# Autodesk Inventor assembly: Base
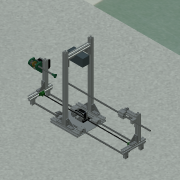
[picture p0: Inventor's stored thumbnail of the model, 180x180]
Saved by Autodesk Inventor 2015 (Build 190159000, 159)
## iProperties
Created: 2015-02-24
Part Number: Base
Document SubType Name: Assembly
Designer: Andrew
Author: Andrew
## Documents named in this file (33)
- C:\Users\pltwe4\Documents\model\Base.iam
- C:\Users\pltwe4\Documents\model\Linear Bearing Platform Small.ipt
- C:\Users\pltwe4\Documents\model\Base Plate.ipt
- C:\Users\pltwe4\Documents\model\NEMA 17 Stepper.ipt
- C:\Users\pltwe4\Documents\model\GT2 Pulley.ipt
- C:\Users\pltwe4\Documents\model\Stepper Motor Mount.ipt
- C:\Users\pltwe4\Documents\model\MainRod.ipt
- C:\Users\pltwe4\Documents\model\Linear Rail Shaft Guide.ipt
- C:\Users\pltwe4\Documents\model\Spur Gear.ipt
- C:\Users\pltwe4\Documents\model\Worm Gear.ipt
- C:\Users\pltwe4\Documents\model\20x20 Slotted Extrusion Arm.ipt
- C:\Users\pltwe4\Documents\model\20x20 Slotted Extrusion Tower.ipt
- C:\Users\pltwe4\Documents\model\Corner Brace.ipt
- C:\Users\pltwe4\Documents\model\Stepper Gear Box.ipt
- C:\Users\pltwe4\Documents\model\Bearing.ipt
- C:\Users\pltwe4\Documents\model\20x20 Slotted Extrusion Stationary Arm.ipt
- C:\Users\pltwe4\Documents\model\Clamp Rod.ipt
- C:\Users\pltwe4\Documents\model\Rotational Rod.ipt
- C:\Users\pltwe4\Documents\model\20x20 Slotted Extrusion Base.ipt
- C:\Users\pltwe4\Documents\model\20x20 Slotted Extrusion Source Bracket.ipt
- C:\Users\pltwe4\Documents\model\Cover.ipt
- C:\Users\pltwe4\Documents\model\X-Ray Tube Assy.ipt.iam
- C:\Users\pltwe4\Documents\model\Hand.ipt
- C:\Users\pltwe4\Documents\model\Linear Bearing Adapter Arm.ipt
- C:\Users\pltwe4\Documents\model\20x20 Slotted Extrusion Base2Plate.ipt
- C:\Users\pltwe4\Documents\model\UnNeeded\Corner Brace_MIR.ipt
- C:\Users\pltwe4\Documents\model\Stepper Adapter.ipt
- C:\Users\pltwe4\Documents\model\Stepper Adapter Cap.ipt
- C:\Users\pltwe4\Documents\model\Belt Clamp.ipt
- C:\Users\pltwe4\Documents\model\GT2 Belt Cut.ipt
- C:\Users\pltwe4\Documents\model\Limit Adapter.ipt
- C:\Users\pltwe4\Documents\model\Limit Switch.ipt
- X-Ray Tube Assy.ipt
## Components (194 placed, 31 different names)
1. Linear Bearing Platform Small:1 — Flush:5, Mate:7, Flush:9, Flush:11
2. Linear Bearing Platform Small:2 — Flush:4, Flush:5, Flush:6, Mate:6, Angle:2, Flush:8, Flush:10
3. Linear Bearing Platform Small:3 — Flush:4, Mate:8, Flush:8, Flush:65, Mate:197, Flush:66, Flush:67
4. Linear Bearing Platform Small:4 — Flush:6, Mate:1, Mate:9, Angle:3, Flush:9
5. Base Plate:1 — Flush:1, Flush:2, Flush:3, Mate:1, Angle:2, Angle:3, Flush:10, Flush:11, Flush:40, Flush:42, Mate:123, Flush:43, Mate:153, Flush:56, Flush:57, Flush:58, Mate:172
6. GT2 Pulley:1 — Mate:22, Mate:166, Mate:170, Mate:192, Mate:194
7. MainRod:1 — Mate:6, Mate:7, Mate:10, Flush:16, Mate:12, Flush:24
8. MainRod:2 — Mate:8, Mate:9, Mate:11, Flush:16, Mate:13, Flush:23
9. Linear Rail Shaft Guide:1 — Mate:10, Flush:14, Flush:15, Flush:24, Flush:53
10. Linear Rail Shaft Guide:2 — Mate:11, Flush:14, Flush:15, Flush:31, Mate:47, Mate:48, Flush:52
11. Linear Rail Shaft Guide:3 — Mate:12
12. Linear Rail Shaft Guide:4 — Mate:13, Flush:23, Flush:32, Mate:49, Mate:50
13. Spur Gear:1 — Angle:5, Mate:87, Mate:99, Mate:203
14. Stepper Motor Mount:2 — Mate:40, Mate:41, Mate:42, Angle:5, Mate:53, Mate:54, Mate:55, Mate:79
15. Worm Gear:1 — Mate:201, Flush:68, Mate:203
16. NEMA 17 Stepper:2 — Mate:40, Mate:41, Mate:42, Mate:81, Mate:201, Flush:68
17. 20x20 Slotted Extrusion Arm:1 — Flush:31, Mate:47, Mate:48, Mate:52, Flush:34, Mate:66, Mate:68, Mate:70, Mate:72, Mate:100, Flush:52, Flush:53, Mate:187, Mate:188
18. 20x20 Slotted Extrusion Tower:1 — Mate:52, Flush:34, Mate:53, Mate:54, Mate:55, Mate:65, Mate:67, Mate:69, Mate:71
19. 20x20 Slotted Extrusion Arm:2 — Flush:32, Mate:49, Mate:50, Mate:51, Flush:33, Mate:57, Mate:58, Mate:63, Mate:64, Mate:189, Mate:190
20. 20x20 Slotted Extrusion Tower:2 — Mate:51, Flush:33, Mate:59, Mate:60, Mate:61, Mate:62, Angle:7, Mate:88, Mate:89, Mate:90, Flush:35, Flush:36, Mate:92, Mate:95
21. Corner Brace:1 — Mate:69, Mate:70, Mate:71, Mate:72
22. Corner Brace:2 — Mate:65, Mate:66, Mate:67, Mate:68
23. Corner Brace:3 — Mate:57, Mate:58, Mate:59, Mate:60
24. Corner Brace:4 — Mate:61, Mate:62, Mate:63, Mate:64
25. Linear Bearing Platform Small:5 — Mate:86, Angle:6, Mate:87, Mate:91, Mate:93, Flush:51, Mate:149, Mate:150
26. Linear Rail Shaft Guide:5 — Mate:86, Angle:6, Angle:7, Mate:88, Mate:89, Mate:90, Flush:35, Mate:91, Flush:50
27. Bearing:1 — Mate:82, Mate:195, Mate:202
28. Bearing:2 — Mate:84, Mate:196
29. 20x20 Slotted Extrusion Stationary Arm:1 — Flush:36, Mate:92, Mate:93, Mate:94, Mate:96, Mate:97
30. Corner Brace:5 — Mate:94, Mate:95, Mate:96, Mate:97
31. Clamp Rod:1 — Mate:98, Flush:50, Mate:147, Mate:152
32. Rotational Rod:1 — Mate:98, Mate:99, Flush:37, Mate:100, Mate:146, Mate:148, Mate:196, Mate:202
33. 20x20 Slotted Extrusion Base:1 — Symmetry:2, Flush:39, Flush:40, Mate:135, Mate:137, Flush:59, Mate:155, Mate:157, Mate:158, Mate:162
34. 20x20 Slotted Extrusion Base:2 — Symmetry:2, Flush:39, Mate:107, Flush:41, Mate:134, Flush:59, Mate:154, Mate:160, Mate:161, Mate:163
35. 20x20 Slotted Extrusion Source Bracket:1 — Mate:107, Flush:41, Mate:140, Mate:141, Mate:142, Mate:143, Mate:144, Mate:155
36. Cover:1 — Flush:42, Mate:123, Flush:43
37. Corner Brace:6 — Mate:135, Flush:48, Flush:49, Mate:137
38. Corner Brace:7 — Mate:134, Flush:48, Flush:49, Mate:144
39. X-Ray Tube Assy.ipt:1 [sub-assembly] — Mate:140, Mate:141, Mate:142, Mate:143
40. Hand:1 — Mate:145, Mate:146, Mate:148
41. 20x20 Slotted Extrusion Base2Plate:1 — Flush:54, Mate:153, Flush:55, Flush:58, Mate:154, Mate:159, Mate:164, Flush:63
42. 20x20 Slotted Extrusion Base2Plate:2 — Flush:54, Flush:55, Flush:56, Flush:57, Mate:156, Mate:165, Angle:8
43. Corner Brace:8 — Mate:156, Mate:157, Mate:158, Flush:61
44. Corner Brace:9 — Mate:159, Mate:160, Mate:161, Flush:60
45. Corner Brace_MIR:1 — Flush:61, Mate:162, Mate:165
46. Corner Brace_MIR:2 — Flush:60, Mate:163, Mate:164
47. NEMA 17 Stepper:3 — Mate:166, Mate:169, Mate:173, Mate:174, Mate:175, Mate:186, Flush:63
48. Stepper Motor Mount:3 — Mate:172, Mate:173, Mate:174, Mate:175, Mate:176, Mate:177
49. Stepper Adapter Cap:1 — Mate:178, Mate:179, Mate:181
50. Bearing:3 — Mate:179, Mate:180
51. Stepper Adapter Cap:2 — Mate:185
52. Bearing:4 — Mate:183, Mate:184, Tangent:2
53. Belt Clamp:2 — Mate:189, Mate:190, Flush:64, Mate:193
54. Limit Switch:1 — Mate:198, Mate:199, Mate:200
55. Stepper Gear Box:1 — Mate:79, Mate:81, Mate:82, Mate:84, Flush:37, Mate:195
56. Hand:2 — Mate:145, Mate:147
57. Linear Bearing Adapter Arm:1 — Flush:51, Mate:149, Mate:150
58. Stepper Adapter:1 — Mate:169, Mate:170, Mate:176, Mate:177, Angle:8, Mate:178, Mate:180, Mate:181, Mate:183, Mate:184, Mate:185, Angle:9
59. Belt Clamp:1 — Mate:187, Mate:188, Flush:64, Mate:194
60. Limit — Flush:65, Mate:197, Flush:66, Flush:67, Mate:198, Mate:199, Mate:200
61. GT2 Belt Cut:1 — Mate:191, Mate:192, Mate:193
62. GT2 Belt Cut:2
63. GT2 Belt Cut:3
64. GT2 Belt Cut:4
65. GT2 Belt Cut:5
66. GT2 Belt Cut:6
67. GT2 Belt Cut:7
68. GT2 Belt Cut:8
69. GT2 Belt Cut:9
70. GT2 Belt Cut:10
71. GT2 Belt Cut:11
72. GT2 Belt Cut:12
73. GT2 Belt Cut:13
74. GT2 Belt Cut:14
75. GT2 Belt Cut:15
76. GT2 Belt Cut:16
77. GT2 Belt Cut:17
78. GT2 Belt Cut:18
79. GT2 Belt Cut:19
80. GT2 Belt Cut:20
81. GT2 Belt Cut:21
82. GT2 Belt Cut:22
83. GT2 Belt Cut:23
84. GT2 Belt Cut:24
85. GT2 Belt Cut:25
86. GT2 Belt Cut:26
87. GT2 Belt Cut:27
88. GT2 Belt Cut:28
89. GT2 Belt Cut:29
90. GT2 Belt Cut:30
91. GT2 Belt Cut:31
92. GT2 Belt Cut:32
93. GT2 Belt Cut:33
94. GT2 Belt Cut:34
95. GT2 Belt Cut:35
96. GT2 Belt Cut:36
97. GT2 Belt Cut:37
98. GT2 Belt Cut:38
99. GT2 Belt Cut:39
100. GT2 Belt Cut:40
101. GT2 Belt Cut:41
102. GT2 Belt Cut:42
103. GT2 Belt Cut:43
104. GT2 Belt Cut:44
105. GT2 Belt Cut:45
106. GT2 Belt Cut:46
107. GT2 Belt Cut:47
108. GT2 Belt Cut:48
109. GT2 Belt Cut:49
110. GT2 Belt Cut:50
111. GT2 Belt Cut:51
112. GT2 Belt Cut:52
113. GT2 Belt Cut:53
114. GT2 Belt Cut:54
115. GT2 Belt Cut:55
116. GT2 Belt Cut:56
117. GT2 Belt Cut:57
118. GT2 Belt Cut:58
119. GT2 Belt Cut:59
120. GT2 Belt Cut:60
121. GT2 Belt Cut:61
122. GT2 Belt Cut:62
123. GT2 Belt Cut:63
124. GT2 Belt Cut:64
125. GT2 Belt Cut:65
126. GT2 Belt Cut:66
127. GT2 Belt Cut:67
128. GT2 Belt Cut:68
129. GT2 Belt Cut:69
130. GT2 Belt Cut:70
131. GT2 Belt Cut:71
132. GT2 Belt Cut:72
133. GT2 Belt Cut:73
134. GT2 Belt Cut:74
135. GT2 Belt Cut:75
136. GT2 Belt Cut:76
137. GT2 Belt Cut:77
138. GT2 Belt Cut:78
139. GT2 Belt Cut:79
140. GT2 Belt Cut:80
141. GT2 Belt Cut:81
142. GT2 Belt Cut:82
143. GT2 Belt Cut:83
144. GT2 Belt Cut:84
145. GT2 Belt Cut:85
146. GT2 Belt Cut:86
147. GT2 Belt Cut:87
148. GT2 Belt Cut:88
149. GT2 Belt Cut:89
150. GT2 Belt Cut:90
151. GT2 Belt Cut:91
152. GT2 Belt Cut:92
153. GT2 Belt Cut:93
154. GT2 Belt Cut:94
155. GT2 Belt Cut:95
156. GT2 Belt Cut:96
157. GT2 Belt Cut:97
158. GT2 Belt Cut:98
159. GT2 Belt Cut:99
160. GT2 Belt Cut:100
161. GT2 Belt Cut:101
162. GT2 Belt Cut:102
163. GT2 Belt Cut:103
164. GT2 Belt Cut:104
165. GT2 Belt Cut:105
166. GT2 Belt Cut:106
167. GT2 Belt Cut:107
168. GT2 Belt Cut:108
169. GT2 Belt Cut:109
170. GT2 Belt Cut:110
171. GT2 Belt Cut:111
172. GT2 Belt Cut:112
173. GT2 Belt Cut:113
174. GT2 Belt Cut:114
175. GT2 Belt Cut:115
176. GT2 Belt Cut:116
177. GT2 Belt Cut:117
178. GT2 Belt Cut:118
179. GT2 Belt Cut:119
180. GT2 Belt Cut:120
181. GT2 Belt Cut:121
182. GT2 Belt Cut:122
183. GT2 Belt Cut:123
184. GT2 Belt Cut:124
185. GT2 Belt Cut:125
186. GT2 Belt Cut:126
187. GT2 Belt Cut:127
188. GT2 Belt Cut:128
189. GT2 Belt Cut:129
190. GT2 Belt Cut:130
191. GT2 Belt Cut:131
192. GT2 Belt Cut:132
193. GT2 Belt Cut:133
194. GT2 Belt Cut:134
## Component patterns: (134 elements, first: GT2 Belt Cut:1)
## Relationships (180: Mate 122, Flush 49, Angle 7, Symmetry 1, Tangent 1)
- Flush:1: Base Plate:1
- Flush:2: Base Plate:1
- Flush:3: Base Plate:1
- Flush:4: Linear Bearing Platform Small:2 ↔ Linear Bearing Platform Small:3
- Flush:5: Linear Bearing Platform Small:1 ↔ Linear Bearing Platform Small:2
- Flush:6: Linear Bearing Platform Small:2 ↔ Linear Bearing Platform Small:4
- Mate:1: Linear Bearing Platform Small:4 ↔ Base Plate:1
- Mate:6: Linear Bearing Platform Small:2 ↔ MainRod:1
- Mate:7: Linear Bearing Platform Small:1 ↔ MainRod:1
- Mate:8: Linear Bearing Platform Small:3 ↔ MainRod:2
- Mate:9: Linear Bearing Platform Small:4 ↔ MainRod:2
- Mate:10: MainRod:1 ↔ Linear Rail Shaft Guide:1
- Mate:11: MainRod:2 ↔ Linear Rail Shaft Guide:2
- Angle:2 (0 deg): Linear Bearing Platform Small:2 ↔ Base Plate:1
- Angle:3 (0 deg): Linear Bearing Platform Small:4 ↔ Base Plate:1
- Flush:8: Linear Bearing Platform Small:2 ↔ Linear Bearing Platform Small:3
- Flush:9: Linear Bearing Platform Small:1 ↔ Linear Bearing Platform Small:4
- Flush:10 (5 mm): Linear Bearing Platform Small:2 ↔ Base Plate:1
- Flush:11 (5 mm): Linear Bearing Platform Small:1 ↔ Base Plate:1
- Flush:14: Linear Rail Shaft Guide:1 ↔ Linear Rail Shaft Guide:2
- Flush:15: Linear Rail Shaft Guide:1 ↔ Linear Rail Shaft Guide:2
- Flush:16: MainRod:1 ↔ MainRod:2
- [Flush]: Linear Rail Shaft Guide:3 ↔ Linear Rail Shaft Guide:4
- [Flush]: Linear Rail Shaft Guide:3 ↔ Linear Rail Shaft Guide:4
- Mate:12: MainRod:1 ↔ Linear Rail Shaft Guide:3
- Mate:13: MainRod:2 ↔ Linear Rail Shaft Guide:4
- Flush:23 (5 mm): MainRod:2 ↔ Linear Rail Shaft Guide:4
- Flush:24 (5 mm): MainRod:1 ↔ Linear Rail Shaft Guide:1
- Mate:22: GT2 Pulley:1
- Mate:40: Stepper Motor Mount:2 ↔ NEMA 17 Stepper:2
- Mate:41: Stepper Motor Mount:2 ↔ NEMA 17 Stepper:2
- Mate:42: Stepper Motor Mount:2 ↔ NEMA 17 Stepper:2
- Angle:5 (0 deg): Spur Gear:1 ↔ Stepper Motor Mount:2
- Flush:31: Linear Rail Shaft Guide:2 ↔ 20x20 Slotted Extrusion Arm:1
- Mate:47: Linear Rail Shaft Guide:2 ↔ 20x20 Slotted Extrusion Arm:1
- Mate:48: Linear Rail Shaft Guide:2 ↔ 20x20 Slotted Extrusion Arm:1
- Flush:32: Linear Rail Shaft Guide:4 ↔ 20x20 Slotted Extrusion Arm:2
- Mate:49: Linear Rail Shaft Guide:4 ↔ 20x20 Slotted Extrusion Arm:2
- Mate:50: Linear Rail Shaft Guide:4 ↔ 20x20 Slotted Extrusion Arm:2
- Mate:51: 20x20 Slotted Extrusion Arm:2 ↔ 20x20 Slotted Extrusion Tower:2
- Flush:33: 20x20 Slotted Extrusion Arm:2 ↔ 20x20 Slotted Extrusion Tower:2
- Mate:52: 20x20 Slotted Extrusion Arm:1 ↔ 20x20 Slotted Extrusion Tower:1
- Flush:34: 20x20 Slotted Extrusion Arm:1 ↔ 20x20 Slotted Extrusion Tower:1
- Mate:53: Stepper Motor Mount:2 ↔ 20x20 Slotted Extrusion Tower:1
- Mate:54: Stepper Motor Mount:2 ↔ 20x20 Slotted Extrusion Tower:1
- Mate:55: Stepper Motor Mount:2 ↔ 20x20 Slotted Extrusion Tower:1
- Mate:57: 20x20 Slotted Extrusion Arm:2 ↔ Corner Brace:3
- Mate:58: 20x20 Slotted Extrusion Arm:2 ↔ Corner Brace:3
- Mate:59: 20x20 Slotted Extrusion Tower:2 ↔ Corner Brace:3
- Mate:60: 20x20 Slotted Extrusion Tower:2 ↔ Corner Brace:3
- Mate:61: 20x20 Slotted Extrusion Tower:2 ↔ Corner Brace:4
- Mate:62: 20x20 Slotted Extrusion Tower:2 ↔ Corner Brace:4
- Mate:63: 20x20 Slotted Extrusion Arm:2 ↔ Corner Brace:4
- Mate:64: 20x20 Slotted Extrusion Arm:2 ↔ Corner Brace:4
- Mate:65: 20x20 Slotted Extrusion Tower:1 ↔ Corner Brace:2
- Mate:66: 20x20 Slotted Extrusion Arm:1 ↔ Corner Brace:2
- Mate:67: 20x20 Slotted Extrusion Tower:1 ↔ Corner Brace:2
- Mate:68: 20x20 Slotted Extrusion Arm:1 ↔ Corner Brace:2
- Mate:69: 20x20 Slotted Extrusion Tower:1 ↔ Corner Brace:1
- Mate:70: 20x20 Slotted Extrusion Arm:1 ↔ Corner Brace:1
- Mate:71: 20x20 Slotted Extrusion Tower:1 ↔ Corner Brace:1
- Mate:72: 20x20 Slotted Extrusion Arm:1 ↔ Corner Brace:1
- Mate:79: Stepper Motor Mount:2 ↔ Stepper Gear Box:1
- Mate:81: NEMA 17 Stepper:2 ↔ Stepper Gear Box:1
- Mate:82: Bearing:1 ↔ Stepper Gear Box:1
- Mate:84: Bearing:2 ↔ Stepper Gear Box:1
- Mate:86: Linear Bearing Platform Small:5 ↔ Linear Rail Shaft Guide:5
- Angle:6 (0 deg): Linear Bearing Platform Small:5 ↔ Linear Rail Shaft Guide:5
- Angle:7 (0 deg): 20x20 Slotted Extrusion Tower:2 ↔ Linear Rail Shaft Guide:5
- Mate:87: Spur Gear:1 ↔ Linear Bearing Platform Small:5
- Mate:88: 20x20 Slotted Extrusion Tower:2 ↔ Linear Rail Shaft Guide:5
- Mate:89: 20x20 Slotted Extrusion Tower:2 ↔ Linear Rail Shaft Guide:5
- Mate:90: 20x20 Slotted Extrusion Tower:2 ↔ Linear Rail Shaft Guide:5
- Flush:35 (-5 mm): 20x20 Slotted Extrusion Tower:2 ↔ Linear Rail Shaft Guide:5
- Mate:91 (50 mm): Linear Bearing Platform Small:5 ↔ Linear Rail Shaft Guide:5
- Flush:36: 20x20 Slotted Extrusion Tower:2 ↔ 20x20 Slotted Extrusion Stationary Arm:1
- Mate:92: 20x20 Slotted Extrusion Tower:2 ↔ 20x20 Slotted Extrusion Stationary Arm:1
- Mate:93: Linear Bearing Platform Small:5 ↔ 20x20 Slotted Extrusion Stationary Arm:1
- Mate:94: 20x20 Slotted Extrusion Stationary Arm:1 ↔ Corner Brace:5
- Mate:95: 20x20 Slotted Extrusion Tower:2 ↔ Corner Brace:5
- Mate:96: 20x20 Slotted Extrusion Stationary Arm:1 ↔ Corner Brace:5
- Mate:97: 20x20 Slotted Extrusion Stationary Arm:1 ↔ Corner Brace:5
- Mate:98: Clamp Rod:1 ↔ Rotational Rod:1
- Mate:99: Spur Gear:1 ↔ Rotational Rod:1
- Flush:37 (-5 mm): Rotational Rod:1 ↔ Stepper Gear Box:1
- Mate:100: 20x20 Slotted Extrusion Arm:1 ↔ Rotational Rod:1
- Symmetry:2: 20x20 Slotted Extrusion Base:1 ↔ 20x20 Slotted Extrusion Base:2
- Flush:39: 20x20 Slotted Extrusion Base:1 ↔ 20x20 Slotted Extrusion Base:2
- Flush:40: Base Plate:1 ↔ 20x20 Slotted Extrusion Base:1
- Mate:107: 20x20 Slotted Extrusion Base:2 ↔ 20x20 Slotted Extrusion Source Bracket:1
- Flush:41: 20x20 Slotted Extrusion Base:2 ↔ 20x20 Slotted Extrusion Source Bracket:1
- Flush:42: Base Plate:1 ↔ Cover:1
- Mate:123: Base Plate:1 ↔ Cover:1
- Flush:43: Base Plate:1 ↔ Cover:1
- Mate:134: 20x20 Slotted Extrusion Base:2 ↔ Corner Brace:7
- Mate:135: 20x20 Slotted Extrusion Base:1 ↔ Corner Brace:6
- Flush:48: Corner Brace:6 ↔ Corner Brace:7
- Flush:49: Corner Brace:6 ↔ Corner Brace:7
- Mate:137: 20x20 Slotted Extrusion Base:1 ↔ Corner Brace:6
- Mate:140: 20x20 Slotted Extrusion Source Bracket:1 ↔ X-Ray Tube Assy.ipt:1
- Mate:141: 20x20 Slotted Extrusion Source Bracket:1 ↔ X-Ray Tube Assy.ipt:1
- Mate:142: 20x20 Slotted Extrusion Source Bracket:1 ↔ X-Ray Tube Assy.ipt:1
- Mate:143: 20x20 Slotted Extrusion Source Bracket:1 ↔ X-Ray Tube Assy.ipt:1
- Mate:144: 20x20 Slotted Extrusion Source Bracket:1 ↔ Corner Brace:7
- Flush:50 (100 mm): Linear Rail Shaft Guide:5 ↔ Clamp Rod:1
- Mate:145: Hand:1 ↔ Hand:2
- Mate:146: Rotational Rod:1 ↔ Hand:1
- Mate:147: Clamp Rod:1 ↔ Hand:2
- Mate:148: Rotational Rod:1 ↔ Hand:1
- Flush:51: Linear Bearing Platform Small:5 ↔ Linear Bearing Adapter Arm:1
- Mate:149: Linear Bearing Platform Small:5 ↔ Linear Bearing Adapter Arm:1
- Mate:150: Linear Bearing Platform Small:5 ↔ Linear Bearing Adapter Arm:1
- Flush:52: Linear Rail Shaft Guide:2 ↔ 20x20 Slotted Extrusion Arm:1
- Flush:53: Linear Rail Shaft Guide:1 ↔ 20x20 Slotted Extrusion Arm:1
- Mate:152: Clamp Rod:1
- Flush:54: 20x20 Slotted Extrusion Base2Plate:1 ↔ 20x20 Slotted Extrusion Base2Plate:2
- Mate:153: Base Plate:1 ↔ 20x20 Slotted Extrusion Base2Plate:1
- Flush:55: 20x20 Slotted Extrusion Base2Plate:1 ↔ 20x20 Slotted Extrusion Base2Plate:2
- Flush:56: Base Plate:1 ↔ 20x20 Slotted Extrusion Base2Plate:2
- Flush:57: Base Plate:1 ↔ 20x20 Slotted Extrusion Base2Plate:2
- Flush:58: Base Plate:1 ↔ 20x20 Slotted Extrusion Base2Plate:1
- Flush:59: 20x20 Slotted Extrusion Base:1 ↔ 20x20 Slotted Extrusion Base:2
- Mate:154: 20x20 Slotted Extrusion Base:2 ↔ 20x20 Slotted Extrusion Base2Plate:1
- Mate:155: 20x20 Slotted Extrusion Base:1 ↔ 20x20 Slotted Extrusion Source Bracket:1
- Mate:156: 20x20 Slotted Extrusion Base2Plate:2 ↔ Corner Brace:8
- Mate:157: 20x20 Slotted Extrusion Base:1 ↔ Corner Brace:8
- Mate:158: 20x20 Slotted Extrusion Base:1 ↔ Corner Brace:8
- Mate:159: 20x20 Slotted Extrusion Base2Plate:1 ↔ Corner Brace:9
- Mate:160: 20x20 Slotted Extrusion Base:2 ↔ Corner Brace:9
- Mate:161: 20x20 Slotted Extrusion Base:2 ↔ Corner Brace:9
- Flush:60: Corner Brace:9 ↔ Corner Brace_MIR:2
- Flush:61: Corner Brace:8 ↔ Corner Brace_MIR:1
- Mate:162: 20x20 Slotted Extrusion Base:1 ↔ Corner Brace_MIR:1
- Mate:163: 20x20 Slotted Extrusion Base:2 ↔ Corner Brace_MIR:2
- Mate:164: 20x20 Slotted Extrusion Base2Plate:1 ↔ Corner Brace_MIR:2
- Mate:165: 20x20 Slotted Extrusion Base2Plate:2 ↔ Corner Brace_MIR:1
- Mate:166: GT2 Pulley:1 ↔ NEMA 17 Stepper:3
- Mate:169: NEMA 17 Stepper:3 ↔ Stepper Adapter:1
- Mate:170: GT2 Pulley:1 ↔ Stepper Adapter:1
- Mate:172: Base Plate:1 ↔ Stepper Motor Mount:3
- Mate:173: NEMA 17 Stepper:3 ↔ Stepper Motor Mount:3
- Mate:174: NEMA 17 Stepper:3 ↔ Stepper Motor Mount:3
- Mate:175: NEMA 17 Stepper:3 ↔ Stepper Motor Mount:3
- Mate:176: Stepper Motor Mount:3 ↔ Stepper Adapter:1
- Mate:177: Stepper Motor Mount:3 ↔ Stepper Adapter:1
- Angle:8 (0 deg): 20x20 Slotted Extrusion Base2Plate:2 ↔ Stepper Adapter:1
- Mate:178: Stepper Adapter Cap:1 ↔ Stepper Adapter:1
- Mate:179: Stepper Adapter Cap:1 ↔ Bearing:3
- Mate:180: Bearing:3 ↔ Stepper Adapter:1
- Mate:181: Stepper Adapter Cap:1 ↔ Stepper Adapter:1
- [Mate]: Stepper Adapter Cap:2 ↔ Bearing:4
- Mate:183: Bearing:4 ↔ Stepper Adapter:1
- Mate:184: Bearing:4 ↔ Stepper Adapter:1
- Mate:185: Stepper Adapter Cap:2 ↔ Stepper Adapter:1
- Mate:186: NEMA 17 Stepper:3
- Flush:63 (50 mm): 20x20 Slotted Extrusion Base2Plate:1 ↔ NEMA 17 Stepper:3
- Angle:9 (0 deg): Stepper Adapter:1
- Tangent:2: Bearing:4
- Mate:187: 20x20 Slotted Extrusion Arm:1 ↔ Belt Clamp:1
- Mate:188: 20x20 Slotted Extrusion Arm:1 ↔ Belt Clamp:1
- Mate:189: 20x20 Slotted Extrusion Arm:2 ↔ Belt Clamp:2
- Mate:190: 20x20 Slotted Extrusion Arm:2 ↔ Belt Clamp:2
- Flush:64: Belt Clamp:2 ↔ Belt Clamp:1
- Mate:191: GT2 Belt Cut:1
- Mate:192: GT2 Pulley:1 ↔ GT2 Belt Cut:1
- Mate:193: Belt Clamp:2 ↔ GT2 Belt Cut:1
- Mate:194: GT2 Pulley:1 ↔ Belt Clamp:1
- Flush:65: Linear Bearing Platform Small:3 ↔ Limit
- Mate:195: Bearing:1 ↔ Stepper Gear Box:1
- Mate:196: Bearing:2 ↔ Rotational Rod:1
- Mate:197: Linear Bearing Platform Small:3 ↔ Limit
- Flush:66: Linear Bearing Platform Small:3 ↔ Limit
- Flush:67: Linear Bearing Platform Small:3 ↔ Limit
- Mate:198: Limit Switch:1 ↔ Limit
- Mate:199: Limit Switch:1 ↔ Limit
- Mate:200: Limit Switch:1 ↔ Limit
- Mate:201: Worm Gear:1 ↔ NEMA 17 Stepper:2
- Flush:68: Worm Gear:1 ↔ NEMA 17 Stepper:2
- Mate:202: Bearing:1 ↔ Rotational Rod:1
- Mate:203: Spur Gear:1 ↔ Worm Gear:1
## Named parameters: d31_d27 = 0 mm, d32_d28 = 0 mm, d285_d282 = 0 mm
